# Autodesk Inventor assembly: Assembly21
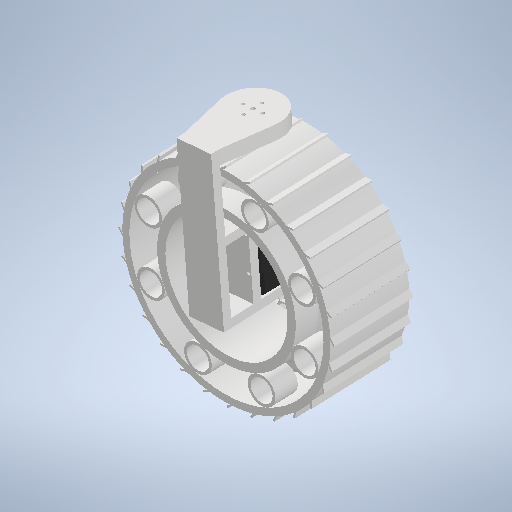
[picture p0: Inventor's stored thumbnail of the model, 512x512]
Saved by Autodesk Inventor 2025.3 (Build 293356000, 356)
## iProperties
Created: 2026-03-13
Part Number: Assembly21
Document SubType Name: Assembly
Designer: ksawe
Author: ksawe
## Documents named in this file (4)
- C:\Users\ksawe\OneDrive\Pulpit\Exomy v1\Assembly21.iam
- C:\Users\ksawe\OneDrive\Pulpit\Exomy v1\felga.ipt
- C:\Users\ksawe\OneDrive\Pulpit\Exomy v1\opona.ipt
- C:\Users\ksawe\OneDrive\Pulpit\Exomy v1\wahaczserwo.iam
## Components (3 placed, 3 different names)
1. felga:1 — Insert:1, Rotational:1
2. opona:1 — Insert:1
3. wahaczserwo:1 [sub-assembly] — Rotational:1
## Relationships (2: Insert 1, RevoluteJoint 1)
- Insert:1: felga:1 ↔ opona:1
- Rotational:1 [RevoluteJoint]: felga:1 ↔ wahaczserwo:1
